# Autodesk Inventor assembly: base
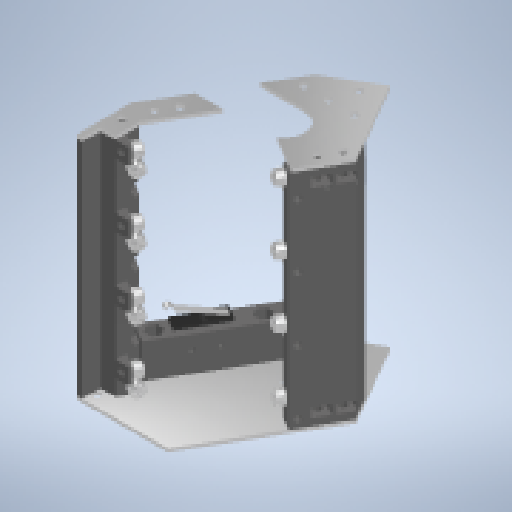
[picture p0: Inventor's stored thumbnail of the model, 512x512]
Saved by Autodesk Inventor 2024.1 (Build 281209000, 209)
## iProperties
Created: 2025-01-17
Part Number: base
Document SubType Name: Assembly
Designer: hibik
Author: hibik
## Documents named in this file (8)
- C:\Users\hibik\Documents\Robomech\RESCUE\ORCA\hard\fork\right\base.iam
- C:\Users\hibik\Documents\Robomech\RESCUE\ORCA\hard\fork\right\base_base.ipt
- C:\Users\hibik\Documents\Robomech\RESCUE\ORCA\hard\fork\right\base_bearingpole_front.ipt
- C:\Users\hibik\Documents\Robomech\RESCUE\ORCA\hard\std_parts\bearing_3_6_2.5.ipt
- C:\Users\hibik\Documents\Robomech\RESCUE\ORCA\hard\fork\right\base_bearingpole_side.ipt
- C:\Users\hibik\Documents\Robomech\RESCUE\ORCA\hard\fork\right\base_cover.ipt
- C:\Users\hibik\Documents\Robomech\RESCUE\ORCA\hard\fork\right\limit_setter_under.ipt
- C:\Users\hibik\Documents\Robomech\RESCUE\ORCA\hard\std_parts\limit_switch.ipt
## Components (23 placed, 7 different names)
1. base_base:1 — メイト:1, フラッシュ:1, フラッシュ:2, メイト:2, フラッシュ:3, フラッシュ:4, フラッシュ:5, フラッシュ:6, フラッシュ:7, メイト:4
2. base_bearingpole_front:1 — メイト:1, フラッシュ:1, フラッシュ:2, 挿入:1, 挿入:2, 挿入:3, 挿入:4, 挿入:5, 挿入:6, 挿入:7, 挿入:8, メイト:5
3. bearing_3_6_2.5:1 — 挿入:1
4. bearing_3_6_2.5:2 — 挿入:2
5. bearing_3_6_2.5:3 — 挿入:3
6. bearing_3_6_2.5:4 — 挿入:4
7. bearing_3_6_2.5:5 — 挿入:5
8. bearing_3_6_2.5:6 — 挿入:6
9. bearing_3_6_2.5:7 — 挿入:7
10. bearing_3_6_2.5:8 — 挿入:8
11. base_bearingpole_side:1 — メイト:2, フラッシュ:3, フラッシュ:4, 挿入:9, 挿入:10, 挿入:11, 挿入:12, 挿入:13, 挿入:14, 挿入:15, 挿入:16, メイト:3, 挿入:19, 挿入:20
12. bearing_3_6_2.5:9 — 挿入:9
13. bearing_3_6_2.5:10 — 挿入:10
14. bearing_3_6_2.5:11 — 挿入:11
15. bearing_3_6_2.5:12 — 挿入:12
16. bearing_3_6_2.5:13 — 挿入:13
17. bearing_3_6_2.5:14 — 挿入:14
18. bearing_3_6_2.5:15 — 挿入:15
19. bearing_3_6_2.5:16 — 挿入:16
20. base_cover:1 — メイト:3, フラッシュ:5, フラッシュ:6
21. limit_setter_under:1 — フラッシュ:7, メイト:4, メイト:5, 挿入:17, 挿入:18
22. limit_switch:1 — 挿入:17, 挿入:18
23. limit_switch:2 — 挿入:19, 挿入:20
## Relationships (32: Insert 20, Flush 7, Mate 5)
- メイト:1 [Mate]: base_base:1 ↔ base_bearingpole_front:1
- フラッシュ:1 [Flush]: base_base:1 ↔ base_bearingpole_front:1
- フラッシュ:2 [Flush]: base_base:1 ↔ base_bearingpole_front:1
- 挿入:1 [Insert]: base_bearingpole_front:1 ↔ bearing_3_6_2.5:1
- 挿入:2 [Insert]: base_bearingpole_front:1 ↔ bearing_3_6_2.5:2
- 挿入:3 [Insert]: base_bearingpole_front:1 ↔ bearing_3_6_2.5:3
- 挿入:4 [Insert]: base_bearingpole_front:1 ↔ bearing_3_6_2.5:4
- 挿入:5 [Insert]: base_bearingpole_front:1 ↔ bearing_3_6_2.5:5
- 挿入:6 [Insert]: base_bearingpole_front:1 ↔ bearing_3_6_2.5:6
- 挿入:7 [Insert]: base_bearingpole_front:1 ↔ bearing_3_6_2.5:7
- 挿入:8 [Insert]: base_bearingpole_front:1 ↔ bearing_3_6_2.5:8
- メイト:2 [Mate]: base_base:1 ↔ base_bearingpole_side:1
- フラッシュ:3 [Flush]: base_base:1 ↔ base_bearingpole_side:1
- フラッシュ:4 [Flush]: base_base:1 ↔ base_bearingpole_side:1
- 挿入:9 [Insert]: base_bearingpole_side:1 ↔ bearing_3_6_2.5:9
- 挿入:10 [Insert]: base_bearingpole_side:1 ↔ bearing_3_6_2.5:10
- 挿入:11 [Insert]: base_bearingpole_side:1 ↔ bearing_3_6_2.5:11
- 挿入:12 [Insert]: base_bearingpole_side:1 ↔ bearing_3_6_2.5:12
- 挿入:13 [Insert]: base_bearingpole_side:1 ↔ bearing_3_6_2.5:13
- 挿入:14 [Insert]: base_bearingpole_side:1 ↔ bearing_3_6_2.5:14
- 挿入:15 [Insert]: base_bearingpole_side:1 ↔ bearing_3_6_2.5:15
- 挿入:16 [Insert]: base_bearingpole_side:1 ↔ bearing_3_6_2.5:16
- メイト:3 [Mate]: base_bearingpole_side:1 ↔ base_cover:1
- フラッシュ:5 [Flush]: base_base:1 ↔ base_cover:1
- フラッシュ:6 [Flush]: base_base:1 ↔ base_cover:1
- フラッシュ:7 [Flush]: base_base:1 ↔ limit_setter_under:1
- メイト:4 [Mate]: base_base:1 ↔ limit_setter_under:1
- メイト:5 [Mate] (1 mm): base_bearingpole_front:1 ↔ limit_setter_under:1
- 挿入:17 [Insert]: limit_setter_under:1 ↔ limit_switch:1
- 挿入:18 [Insert]: limit_setter_under:1 ↔ limit_switch:1
- 挿入:19 [Insert]: base_bearingpole_side:1 ↔ limit_switch:2
- 挿入:20 [Insert]: base_bearingpole_side:1 ↔ limit_switch:2
